# Autodesk Inventor assembly: Assembly 2
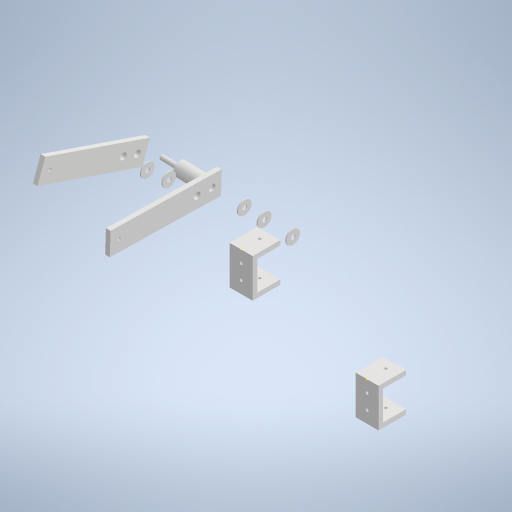
[picture p0: Inventor's stored thumbnail of the model, 512x512]
Saved by Autodesk Inventor 2023 (Build 270158000, 158)
## iProperties
Created: 2022-06-16
Part Number: Assembly 2
Document SubType Name: Assembly
Designer: chait
Author: chait
## Documents named in this file (6)
- D:\Assembly 2.iam
- D:\Screw 5 mm.ipt
- D:\spacer.ipt
- D:\Stationary arm 2.ipt
- D:\Nylon rod.ipt
- D:\clamp.ipt
## Components (13 placed, 5 different names)
1. Screw 5 mm:1 — Mate:1, Flush:1, Mate:2, Mate:3, Mate:4, Mate:5, Mate:6, Mate:7, Mate:8, Mate:9, Mate:10, Mate:11
2. spacer:1
3. spacer:2 — Mate:3, Mate:5, Mate:6, Flush:3, Flush:4
4. spacer:3 — Mate:1, Flush:1, Flush:2, Flush:3
5. spacer:4 — Mate:9
6. spacer:5 — Mate:7
7. spacer:6 — Mate:10
8. spacer:7
9. Stationary arm 2:1 — Mate:2, Flush:2
10. Stationary arm 2:2 — Mate:11
11. Nylon rod:1 — Mate:4, Mate:8, Flush:4
12. clamp:1
13. clamp:2
## Relationships (15: Mate 11, Flush 4)
- Mate:1: Screw 5 mm:1 ↔ spacer:3
- Flush:1: Screw 5 mm:1 ↔ spacer:3
- Mate:2: Screw 5 mm:1 ↔ Stationary arm 2:1
- Flush:2: spacer:3 ↔ Stationary arm 2:1
- Mate:3: Screw 5 mm:1 ↔ spacer:2
- Mate:4: Screw 5 mm:1 ↔ Nylon rod:1
- Mate:5: Screw 5 mm:1 ↔ spacer:2
- Mate:6: Screw 5 mm:1 ↔ spacer:2
- Mate:7: Screw 5 mm:1 ↔ spacer:5
- Mate:8: Screw 5 mm:1 ↔ Nylon rod:1
- Mate:9: Screw 5 mm:1 ↔ spacer:4
- Mate:10: Screw 5 mm:1 ↔ spacer:6
- Mate:11: Screw 5 mm:1 ↔ Stationary arm 2:2
- Flush:3: spacer:2 ↔ spacer:3
- Flush:4: spacer:2 ↔ Nylon rod:1
